# Autodesk Inventor assembly: TorsoSideUnit
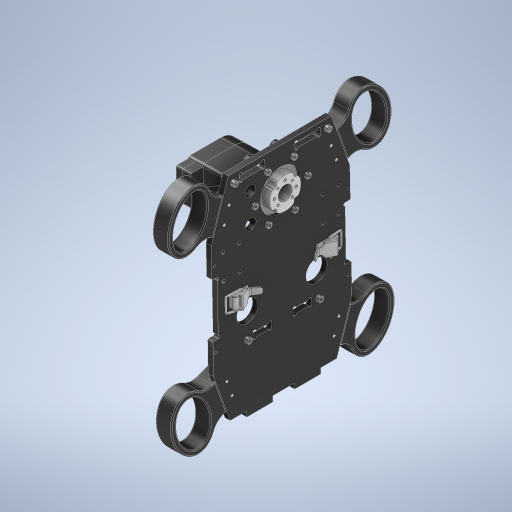
[picture p0: Inventor's stored thumbnail of the model, 512x512]
Saved by Autodesk Inventor 2024.2 (Build 282272000, 272)
## iProperties
Created: 2024-01-05
Part Number: TorsoSideUnit
Document SubType Name: Assembly
Designer: Masato Kubotera
Mass: 444.057 g
Surface Area: 821.622 cm^2
Volume: 159.843 cm^3
Author: Masato Kubotera
## Documents named in this file (8)
- D:\OneDrive - Chiba Institute of Technology\CIT Brains\RoboCup2024\Mechanic\SUSTAINA-OP2-DEV - 作業\NativeFiles\Boby\Torso\TorsoSideUnit.iam
- D:\OneDrive - Chiba Institute of Technology\CIT Brains\RoboCup2024\Mechanic\SUSTAINA-OP2-DEV - 作業\NativeFiles\Boby\COTS\Screws\CapScrew\UC-0310.ipt
- D:\OneDrive - Chiba Institute of Technology\CIT Brains\RoboCup2024\Mechanic\SUSTAINA-OP2-DEV - 作業\NativeFiles\Boby\COTS\MisumiComponents\PKWS1.iam
- D:\OneDrive - Chiba Institute of Technology\CIT Brains\RoboCup2024\Mechanic\SUSTAINA-OP2-DEV - 作業\NativeFiles\Boby\COTS\Screws\CapScrew\UC-0308.ipt
- D:\OneDrive - Chiba Institute of Technology\CIT Brains\RoboCup2024\Mechanic\SUSTAINA-OP2-DEV - 作業\NativeFiles\Boby\COTS\Screws\LowHeadCapScrew\ULC-0306.ipt
- D:\OneDrive - Chiba Institute of Technology\CIT Brains\RoboCup2024\Mechanic\SUSTAINA-OP2-DEV - 作業\NativeFiles\Boby\UpperLimb\Shoulders\LeftShoulderBearingUnit.iam
- D:\OneDrive - Chiba Institute of Technology\CIT Brains\RoboCup2024\Mechanic\SUSTAINA-OP2-DEV - 作業\NativeFiles\Boby\Torso\TorsoBumpers\UpperBumperUnit.iam
- D:\OneDrive - Chiba Institute of Technology\CIT Brains\RoboCup2024\Mechanic\SUSTAINA-OP2-DEV - 作業\NativeFiles\Boby\Torso\TorsoSideFrame.ipt
## Components (18 placed, 7 different names)
1. LeftShoulderBearingUnit:1 [sub-assembly] — Insert:256, Angle:1
2. UpperBumperUnit:1 [sub-assembly] — Insert:259, Insert:260
3. UpperBumperUnit:2 [sub-assembly] — Insert:257, Insert:258
4. UpperBumperUnit:3 [sub-assembly] — Insert:261, Insert:262
5. UpperBumperUnit:4 [sub-assembly] — Insert:263, Insert:264
6. PKWS1:1 [sub-assembly] — Insert:23, Insert:24
7. PKWS1:2 [sub-assembly] — Insert:25, Insert:26
8. TorsoSideFrame:1 — Insert:21, Insert:22, Insert:23, Insert:24, Insert:25, Insert:26, Insert:166, Insert:167, Insert:255, Insert:256, Insert:257, Insert:258, Insert:259, Insert:260, Insert:261, Insert:262, Insert:263, Insert:264
9. UC-0308:8 — Insert:166
10. UC-0308:7 — Insert:167
11. UC-0310:2 — Insert:22
12. UC-0310:1 — Insert:21
13. ULC-0306:1 — Insert:255
14. ULC-0306:2
15. ULC-0306:3
16. ULC-0306:4
17. ULC-0306:5
18. ULC-0306:6
## Component patterns: (6 elements, first: ULC-0306:1)
## Relationships (19: Insert 18, Angle 1)
- Insert:21: TorsoSideFrame:1 ↔ UC-0310:1
- Insert:22: TorsoSideFrame:1 ↔ UC-0310:2
- Insert:23: PKWS1:1 ↔ TorsoSideFrame:1
- Insert:24: PKWS1:1 ↔ TorsoSideFrame:1
- Insert:25: PKWS1:2 ↔ TorsoSideFrame:1
- Insert:26: PKWS1:2 ↔ TorsoSideFrame:1
- Insert:166: TorsoSideFrame:1 ↔ UC-0308:8
- Insert:167: TorsoSideFrame:1 ↔ UC-0308:7
- Insert:255: TorsoSideFrame:1 ↔ ULC-0306:1
- Insert:256: LeftShoulderBearingUnit:1 ↔ TorsoSideFrame:1
- Angle:1 (0 deg): LeftShoulderBearingUnit:1
- Insert:257: UpperBumperUnit:2 ↔ TorsoSideFrame:1
- Insert:258: UpperBumperUnit:2 ↔ TorsoSideFrame:1
- Insert:259: UpperBumperUnit:1 ↔ TorsoSideFrame:1
- Insert:260: UpperBumperUnit:1 ↔ TorsoSideFrame:1
- Insert:261: UpperBumperUnit:3 ↔ TorsoSideFrame:1
- Insert:262: UpperBumperUnit:3 ↔ TorsoSideFrame:1
- Insert:263: UpperBumperUnit:4 ↔ TorsoSideFrame:1
- Insert:264: UpperBumperUnit:4 ↔ TorsoSideFrame:1
